# Autodesk Inventor assembly: Assembly1
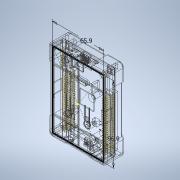
[picture p0: Inventor's stored thumbnail of the model, 180x180]
Saved by Autodesk Inventor 2020 (Build 240168000, 168)
## iProperties
Created: 2025-03-09
Part Number: Assembly1
Document SubType Name: Assembly
Designer: mahun
Author: mahun
## Documents named in this file (4)
- C:\Users\mahun\Desktop\MINBOT LABS\PROJECT\Hoc STM32F411VET6\Case for STM32F4-Discovery Board\Assembly1.iam
- C:\Users\mahun\Desktop\MINBOT LABS\PROJECT\Hoc STM32F411VET6\Case for STM32F4-Discovery Board\case.ipt
- C:\Users\mahun\Desktop\MINBOT LABS\PROJECT\Hoc STM32F411VET6\Case for STM32F4-Discovery Board\stm32f411EDISCO.ipt
- C:\Users\mahun\Desktop\MINBOT LABS\PROJECT\Hoc STM32F411VET6\Case for STM32F4-Discovery Board\nap.ipt
## Components (3 placed, 3 different names)
1. case:1 — Mate:1, Mate:2, Mate:3, Flush:1, Mate:4, Mate:5
2. stm32f411EDISCO:1 — Mate:1, Mate:2, Mate:3
3. nap:1 — Flush:1, Mate:4, Mate:5
## Relationships (6: Mate 5, Flush 1)
- Mate:1: case:1 ↔ stm32f411EDISCO:1
- Mate:2: case:1 ↔ stm32f411EDISCO:1
- Mate:3: case:1 ↔ stm32f411EDISCO:1
- Flush:1: case:1 ↔ nap:1
- Mate:4 (0.1 mm): case:1 ↔ nap:1
- Mate:5 (0.1 mm): case:1 ↔ nap:1
